# Autodesk Inventor assembly: assembly colour sorting machine
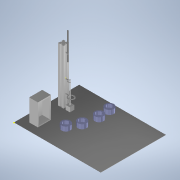
[picture p0: Inventor's stored thumbnail of the model, 180x180]
Saved by Autodesk Inventor 2022 (Build 260153000, 153)
## iProperties
Created: 2022-02-22
Part Number: assembly colour sorting machine
Document SubType Name: Assembly
Designer: admin
Author: admin
## Documents named in this file (10)
- C:\Users\admin\Desktop\assembly colour sorting machine.iam
- D:\canon\sorting machine\Part6.ipt
- D:\canon\sorting machine\part5.ipt
- D:\canon\sorting machine\Part2.ipt
- D:\canon\sorting machine\Part3.ipt
- D:\canon\sorting machine\Part10.ipt
- D:\canon\sorting machine\Part9.ipt
- D:\canon\sorting machine\Part11.ipt
- D:\canon\sorting machine\Part12.ipt
- D:\canon\sorting machine\Part13.ipt
## Components (12 placed, 9 different names)
1. Part6:1 — Mate:1, Mate:2, Mate:4, Mate:5, Mate:6, Mate:12, Mate:13
2. part5:1 — Mate:1, Mate:2, Mate:3
3. Part2:1 — Mate:3
4. Part3:1 — Mate:4, Mate:5
5. Part10:1 — Mate:6, Mate:7, Mate:8, Mate:9, Mate:10, Mate:11, Mate:14
6. Part9:1 — Mate:8
7. Part9:2 — Mate:7
8. Part9:3 — Mate:10
9. Part9:4 — Mate:9
10. Part11:1 — Mate:11
11. Part12:1 — Mate:12, Mate:13
12. Part13:1 — Mate:14
## Relationships (14: Mate 14)
- Mate:1: Part6:1 ↔ part5:1
- Mate:2: Part6:1 ↔ part5:1
- Mate:3: part5:1 ↔ Part2:1
- Mate:4: Part6:1 ↔ Part3:1
- Mate:5: Part6:1 ↔ Part3:1
- Mate:6: Part6:1 ↔ Part10:1
- Mate:7: Part10:1 ↔ Part9:2
- Mate:8: Part10:1 ↔ Part9:1
- Mate:9: Part10:1 ↔ Part9:4
- Mate:10: Part10:1 ↔ Part9:3
- Mate:11: Part10:1 ↔ Part11:1
- Mate:12: Part6:1 ↔ Part12:1
- Mate:13: Part6:1 ↔ Part12:1
- Mate:14: Part10:1 ↔ Part13:1
